# Autodesk Inventor assembly: Transmission Pulley
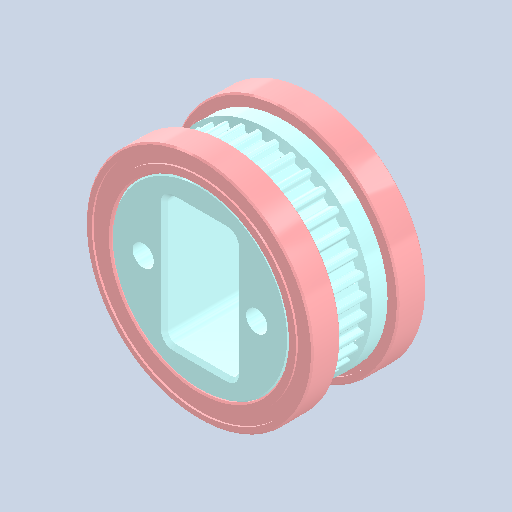
[picture p0: Inventor's stored thumbnail of the model, 512x512]
Saved by Autodesk Inventor 2022.2 (Build 262287000, 287)
## iProperties
Created: 2022-01-01
Part Number: Transmission Pulley
Document SubType Name: Assembly
Designer: Jochen
Author: Jochen
## Documents named in this file (3)
- D:\Projects\Chewbacca\CAD\Common\Motor\Transmission Pulley.iam
- D:\Projects\Chewbacca\CAD\Common\Motor\TransmissionPulleyOutput.ipt
- D:\Projects\Chewbacca\CAD\Common\Motor\bearing_32_25_4_sbn_61705RS.ipt
## Components (3 placed, 2 different names)
1. TransmissionPulleyOutput:1 — Mate:1, Mate:2, Mate:3, Mate:4
2. bearing_32_25_4_sbn_61705RS:1 — Mate:1, Mate:4
3. bearing_32_25_4_sbn_61705RS:2 — Mate:2, Mate:3
## Relationships (4: Mate 4)
- Mate:1: TransmissionPulleyOutput:1 ↔ bearing_32_25_4_sbn_61705RS:1
- Mate:2: TransmissionPulleyOutput:1 ↔ bearing_32_25_4_sbn_61705RS:2
- Mate:3: TransmissionPulleyOutput:1 ↔ bearing_32_25_4_sbn_61705RS:2
- Mate:4: TransmissionPulleyOutput:1 ↔ bearing_32_25_4_sbn_61705RS:1
